# Autodesk Inventor assembly: pcb_test_fitting
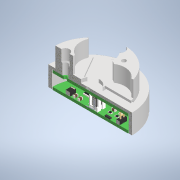
[picture p0: Inventor's stored thumbnail of the model, 180x180]
Saved by Autodesk Inventor 2020.2 (Build 242310000, 310)
## iProperties
Created: 2022-09-19
Part Number: pcb_test_fitting
Document SubType Name: Assembly
Designer: g.schardt
Author: g.schardt
## Documents named in this file (4)
- C:\Users\g.schardt\Inventor\Tauchlampe\pcb_test_fitting.iam
- C:\Users\g.schardt\Inventor\Tauchlampe\akkuhalterung_deckel_2.ipt
- C:\Users\g.schardt\Inventor\Tauchlampe\PCBs\batteriedeckel.iam
- C:\Users\g.schardt\Inventor\Tauchlampe\PCBs\led_buck_3a.iam
## Components (3 placed, 3 different names)
1. akkuhalterung_deckel_2:1 — Passend:1, Passend:2, Passend:3
2. batteriedeckel:1 [sub-assembly] — Passend:1, Passend:2, Passend:3, Passend:4, Passend:5, Passend:6
3. led_buck_3a:1 [sub-assembly] — Passend:4, Passend:5, Passend:6
## Relationships (6: Mate 6)
- Passend:1 [Mate]: akkuhalterung_deckel_2:1 ↔ batteriedeckel:1
- Passend:2 [Mate]: akkuhalterung_deckel_2:1 ↔ batteriedeckel:1
- Passend:3 [Mate]: akkuhalterung_deckel_2:1 ↔ batteriedeckel:1
- Passend:4 [Mate] (7 mm): batteriedeckel:1 ↔ led_buck_3a:1
- Passend:5 [Mate]: batteriedeckel:1 ↔ led_buck_3a:1
- Passend:6 [Mate]: batteriedeckel:1 ↔ led_buck_3a:1
